# Autodesk Inventor assembly: Assembly12
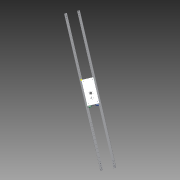
[picture p0: Inventor's stored thumbnail of the model, 180x180]
Saved by Autodesk Inventor 2015 (Build 190159000, 159)
## iProperties
Created: 2015-01-11
Part Number: Assembly12
Document SubType Name: Assembly
Designer: mastkee16
Author: mastkee16
## Documents named in this file (8)
- \\lhssvr02\Homedirs\Robotics Club\CAD Model 2015\claw\Assemblyclaw.iam
- \\lhssvr02\Homedirs\Robotics Club\CAD Model 2015\claw\trolley plate.ipt
- \\lhssvr02\Homedirs\Robotics Club\CAD Model 2015\claw\wheel.ipt
- \\lhssvr02\Homedirs\Robotics Club\CAD Model 2015\claw\.313 peg.ipt
- \\lhssvr02\Homedirs\Robotics Club\CAD Model 2015\claw\c hannel.ipt
- \\lhssvr02\Homedirs\Robotics Club\CAD Model 2015\claw\motor.ipt
- \\lhssvr02\Homedirs\Robotics Club\CAD Model 2015\claw\#6 screw.ipt
- \\lhssvr02\Homedirs\Robotics Club\CAD Model 2015\claw\.25 peg.ipt
## Components (28 placed, 7 different names)
1. trolley plate:1 — Insert:1, Insert:2, Insert:3, Insert:4, Insert:9, Insert:10, Insert:11, Insert:12, Tangent:5, Mate:4
2. wheel:1 — Insert:6, Mate:1, Tangent:2
3. wheel:2 — Insert:5, Tangent:3
4. wheel:3 — Insert:8, Tangent:4, Mate:3
5. wheel:4 — Insert:7, Mate:2, Tangent:1
6. .313 peg:1 — Insert:1, Insert:5
7. .313 peg:2 — Insert:2, Insert:6
8. .313 peg:3 — Insert:3, Insert:8
9. .313 peg:4 — Insert:4, Insert:7
10. c hannel:1 — Tangent:3, Tangent:4, Mate:3, Insert:14, Insert:15, Insert:16, Insert:19, Insert:21, Insert:23
11. c hannel:2 — Mate:1, Mate:2, Tangent:1, Tangent:2, Insert:13, Insert:17, Insert:18, Insert:20, Insert:22, Insert:24
12. motor:1 — Tangent:5, Mate:4
13. #6 screw:1 — Insert:12
14. #6 screw:2 — Insert:9
15. #6 screw:3 — Insert:11
16. #6 screw:4 — Insert:10
17. .25 peg:1 — Insert:24
18. .25 peg:2 — Insert:21
19. .25 peg:3 — Insert:23
20. .25 peg:4 — Insert:19
21. .25 peg:5 — Insert:20
22. .25 peg:6 — Insert:18
23. .25 peg:7 — Insert:17
24. .25 peg:8 — Insert:16
25. .25 peg:9 — Insert:13
26. .25 peg:10 — Insert:22
27. .25 peg:11 — Insert:15
28. .25 peg:12 — Insert:14
## Relationships (33: Insert 24, Tangent 5, Mate 4)
- Insert:1 (-38.1 mm): trolley plate:1 ↔ .313 peg:1
- Insert:2 (-38.1 mm): trolley plate:1 ↔ .313 peg:2
- Insert:3 (-38.1 mm): trolley plate:1 ↔ .313 peg:3
- Insert:4 (-38.1 mm): trolley plate:1 ↔ .313 peg:4
- Insert:5 (-7.747 mm): wheel:2 ↔ .313 peg:1
- Insert:6 (-7.747 mm): wheel:1 ↔ .313 peg:2
- Insert:7 (7.747 mm): wheel:4 ↔ .313 peg:4
- Insert:8 (7.747 mm): wheel:3 ↔ .313 peg:3
- Mate:1: wheel:1 ↔ c hannel:2
- Mate:2: wheel:4 ↔ c hannel:2
- Tangent:1: wheel:4 ↔ c hannel:2
- Tangent:2: wheel:1 ↔ c hannel:2
- Tangent:3: wheel:2 ↔ c hannel:1
- Tangent:4: wheel:3 ↔ c hannel:1
- Mate:3: wheel:3 ↔ c hannel:1
- Insert:9: trolley plate:1 ↔ #6 screw:2
- Insert:10: trolley plate:1 ↔ #6 screw:4
- Insert:11: trolley plate:1 ↔ #6 screw:3
- Insert:12: trolley plate:1 ↔ #6 screw:1
- Tangent:5: trolley plate:1 ↔ motor:1
- Mate:4: trolley plate:1 ↔ motor:1
- Insert:13: c hannel:2 ↔ .25 peg:9
- Insert:14: c hannel:1 ↔ .25 peg:12
- Insert:15: c hannel:1 ↔ .25 peg:11
- Insert:16: c hannel:1 ↔ .25 peg:8
- Insert:17: c hannel:2 ↔ .25 peg:7
- Insert:18: c hannel:2 ↔ .25 peg:6
- Insert:19: c hannel:1 ↔ .25 peg:4
- Insert:20: c hannel:2 ↔ .25 peg:5
- Insert:21: c hannel:1 ↔ .25 peg:2
- Insert:22: c hannel:2 ↔ .25 peg:10
- Insert:23: c hannel:1 ↔ .25 peg:3
- Insert:24: c hannel:2 ↔ .25 peg:1
